# Autodesk Inventor assembly: model-b2 1
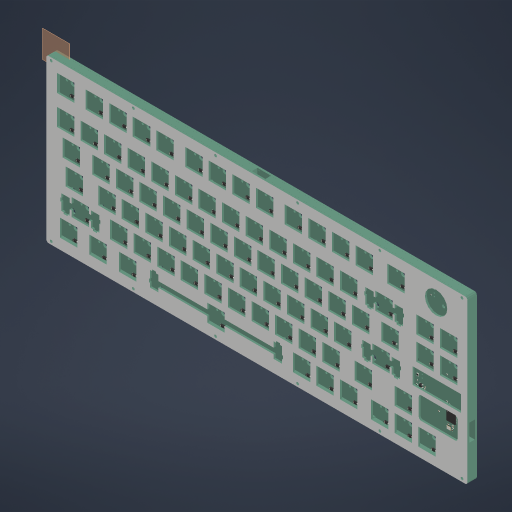
[picture p0: Inventor's stored thumbnail of the model, 512x512]
Saved by Autodesk Inventor 2024.2 (Build 282272000, 272)
## iProperties
Company: Kicad
Created: 2024-07-05
Part Number: model-b2 1
Description: KiCad electronic assembly
Document SubType Name: Assembly
Designer: Moe
Authority: Unknown
Sending System: KiCad to STEP converter
Preprocessor: Open CASCADE STEP processor 7.7
Title: model-b2.step
Author: Pcbnew
## Documents named in this file (11)
- D:\Code\git\Model-B\case\model-b\model-b.iam
- D:\Code\git\Model-B\case\model-b\D_SOD-123.iam
- D:\Code\git\Model-B\case\model-b\C_0402_1005Metric.iam
- D:\Code\git\Model-B\case\model-b\R_0402_1005Metric.iam
- D:\Code\git\Model-B\case\model-b\SOT-23-5.iam
- D:\Code\git\Model-B\case\model-b\QFN-56-1EP_7x7mm_P0.4mm_EP5.6x5.6mm.iam
- D:\Code\git\Model-B\case\model-b\Crystal_SMD_3225-4Pin_3.2x2.5mm.iam
- D:\Code\git\Model-B\case\model-b\Fuse_0805_2012Metric.iam
- D:\Code\git\Model-B\case\model-b\model-b PCB.ipt
- D:\Code\git\Model-B\case\model-b\open_liner.ipt
- D:\Code\git\Model-B\case\model-b\swplate.ipt
## Components (125 placed, 125 different names)
1. 2 [sub-assembly]
2. 4 [sub-assembly]
3. 6 [sub-assembly]
4. 7 [sub-assembly]
5. 8 [sub-assembly]
6. 9 [sub-assembly]
7. 11 [sub-assembly]
8. 12 [sub-assembly]
9. 13 [sub-assembly]
10. 14 [sub-assembly]
11. 15 [sub-assembly]
12. 16 [sub-assembly]
13. 17 [sub-assembly]
14. 18 [sub-assembly]
15. 19 [sub-assembly]
16. 20 [sub-assembly]
17. 21 [sub-assembly]
18. 22 [sub-assembly]
19. 23 [sub-assembly]
20. 24 [sub-assembly]
21. 25 [sub-assembly]
22. 26 [sub-assembly]
23. 27 [sub-assembly]
24. 28 [sub-assembly]
25. 29 [sub-assembly]
26. 30 [sub-assembly]
27. 31 [sub-assembly]
28. 32 [sub-assembly]
29. 33 [sub-assembly]
30. 34 [sub-assembly]
31. 35 [sub-assembly]
32. 36 [sub-assembly]
33. 37 [sub-assembly]
34. 38 [sub-assembly]
35. 39 [sub-assembly]
36. 40 [sub-assembly]
37. 42 [sub-assembly]
38. 43 [sub-assembly]
39. 44 [sub-assembly]
40. 45 [sub-assembly]
41. 46 [sub-assembly]
42. 47 [sub-assembly]
43. 48 [sub-assembly]
44. 49 [sub-assembly]
45. 50 [sub-assembly]
46. 51 [sub-assembly]
47. 52 [sub-assembly]
48. 53 [sub-assembly]
49. 54 [sub-assembly]
50. 55 [sub-assembly]
51. 56 [sub-assembly]
52. 57 [sub-assembly]
53. 58 [sub-assembly]
54. 59 [sub-assembly]
55. 60 [sub-assembly]
56. 61 [sub-assembly]
57. 62 [sub-assembly]
58. 63 [sub-assembly]
59. 64 [sub-assembly]
60. 65 [sub-assembly]
61. 66 [sub-assembly]
62. 67 [sub-assembly]
63. 68 [sub-assembly]
64. 69 [sub-assembly]
65. 70 [sub-assembly]
66. 71 [sub-assembly]
67. 72 [sub-assembly]
68. 73 [sub-assembly]
69. 74 [sub-assembly]
70. 75 [sub-assembly]
71. 76 [sub-assembly]
72. 77 [sub-assembly]
73. 78 [sub-assembly]
74. 79 [sub-assembly]
75. 81 [sub-assembly]
76. 82 [sub-assembly]
77. 83 [sub-assembly]
78. 84 [sub-assembly]
79. 85 [sub-assembly]
80. 86 [sub-assembly]
81. 87 [sub-assembly]
82. 88 [sub-assembly]
83. 89 [sub-assembly]
84. 90 [sub-assembly]
85. 91 [sub-assembly]
86. 92 [sub-assembly]
87. 93 [sub-assembly]
88. 94 [sub-assembly]
89. 95 [sub-assembly]
90. 96 [sub-assembly]
91. 97 [sub-assembly]
92. 98 [sub-assembly]
93. 99 [sub-assembly]
94. 100 [sub-assembly]
95. 101 [sub-assembly]
96. 102 [sub-assembly]
97. 103 [sub-assembly]
98. 104 [sub-assembly]
99. 105 [sub-assembly]
100. 106 [sub-assembly]
101. 107 [sub-assembly]
102. 108 [sub-assembly]
103. 109 [sub-assembly]
104. 110 [sub-assembly]
105. 111 [sub-assembly]
106. 112 [sub-assembly]
107. 113 [sub-assembly]
108. 114 [sub-assembly]
109. 115 [sub-assembly]
110. 116 [sub-assembly]
111. 117 [sub-assembly]
112. 119 [sub-assembly]
113. 120 [sub-assembly]
114. 121 [sub-assembly]
115. 122 [sub-assembly]
116. 123 [sub-assembly]
117. 124 [sub-assembly]
118. 125 [sub-assembly]
119. 126 [sub-assembly]
120. 129 [sub-assembly]
121. 130 [sub-assembly]
122. 131 [sub-assembly]
123. 132 — Mate:1
124. open_liner:1 — Mate:1, Mate:2
125. swplate:1 — Mate:2
## Relationships (2: Mate 2)
- Mate:1: 132 ↔ open_liner:1
- Mate:2: open_liner:1 ↔ swplate:1
## Named parameters: Finish1_Area = 259.807
note: some values were not read from the file. Shown as the stored number, unit unknown: "Finish1_Area".
